# Autodesk Inventor assembly: assembly1'
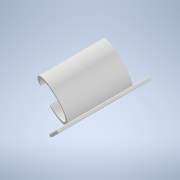
[picture p0: Inventor's stored thumbnail of the model, 180x180]
Saved by Autodesk Inventor 2022 (Build 260153000, 153)
## iProperties
Created: 2021-09-28
Part Number: assembly1'
Document SubType Name: Assembly
Designer: royja
Author: royja
## Documents named in this file (3)
- C:\Users\royja\Dropbox\UCLA_msc_ee\classes\theatre212\augmented flute\3d cad files\assembly1'.iam
- C:\Users\royja\Dropbox\UCLA_msc_ee\classes\theatre212\augmented flute\3d cad files\flute-wrapper.ipt
- C:\Users\royja\Dropbox\UCLA_msc_ee\classes\theatre212\augmented flute\3d cad files\plate4atrduino.ipt
## Components (2 placed, 2 different names)
1. flute-wrapper:1 — Flush:2, Tangent:2, Tangent:3
2. plate4atrduino:1 — Flush:1, Flush:4, Angle:1, Flush:7
## Relationships (8: Flush 4, Tangent 2, Mate 1, Angle 1)
- Flush:1 (-24.5 mm): plate4atrduino:1
- Flush:2 (-17 mm): flute-wrapper:1
- Mate:1
- Flush:4 (-1 mm): plate4atrduino:1
- Angle:1 (0 deg): plate4atrduino:1
- Tangent:2: flute-wrapper:1
- Flush:7: plate4atrduino:1
- Tangent:3: flute-wrapper:1
